# Autodesk Inventor assembly: rimAssembly
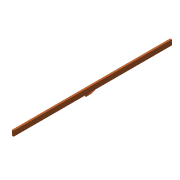
[picture p0: Inventor's stored thumbnail of the model, 180x180]
Saved by Autodesk Inventor 2016 SP2 (Build 200236200, 236)
## iProperties
Created: 2013-12-03
Part Number: rimAssembly
Document SubType Name: Assembly
Designer: Dave
Author: Dave
## Documents named in this file (3)
- C:\Users\krosie\Google Drive\HERA\hera-cad\support\rimAssembly.iam
- C:\Users\krosie\Google Drive\HERA\hera-cad\support\rimHoriz.ipt
- C:\Users\krosie\Google Drive\HERA\hera-cad\support\rimIntermediateSparHolder.ipt
## Components (2 placed, 2 different names)
1. rimHoriz:1 — Insert:2, Insert:3
2. rimIntermediateSparHolder:1 — Insert:2, Insert:3
## Relationships (2: Insert 2)
- Insert:2: rimHoriz:1 ↔ rimIntermediateSparHolder:1
- Insert:3: rimHoriz:1 ↔ rimIntermediateSparHolder:1
